# Autodesk Inventor assembly: Assembly_Doorhinge
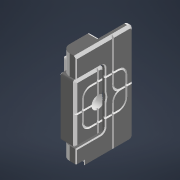
[picture p0: Inventor's stored thumbnail of the model, 180x180]
Saved by Autodesk Inventor 2022.1 (Build 261234000, 234)
## iProperties
Created: 2021-10-11
Part Number: Assembly_Doorhinge
Document SubType Name: Assembly
Designer: Rama
Author: Rama
## Documents named in this file (3)
- C:\Users\Rama\Desktop\GitHub\Voron-2-Mods\Panel_Clips\CAD\Assembly_Doorhinge.iam
- C:\Users\Rama\Desktop\GitHub\Voron-2-Mods\Panel_Clips\CAD\Doorhinge_Outlet.ipt
- C:\Users\Rama\Desktop\GitHub\Voron-2-Mods\Panel_Clips\CAD\Doorhinge_Inlet.ipt
## Components (2 placed, 2 different names)
1. Doorhinge_Outlet:1 — Passend:1, Passend:2, Fluchtend:1, Passend:3
2. Doorhinge_Inlet:1 — Passend:1, Passend:2, Fluchtend:1, Passend:3
## Relationships (4: Mate 3, Flush 1)
- Passend:1 [Mate]: Doorhinge_Outlet:1 ↔ Doorhinge_Inlet:1
- Passend:2 [Mate]: Doorhinge_Outlet:1 ↔ Doorhinge_Inlet:1
- Fluchtend:1 [Flush]: Doorhinge_Outlet:1 ↔ Doorhinge_Inlet:1
- Passend:3 [Mate] (0.4 mm): Doorhinge_Outlet:1 ↔ Doorhinge_Inlet:1
